# Autodesk Inventor assembly: ASY GBK правая стенка
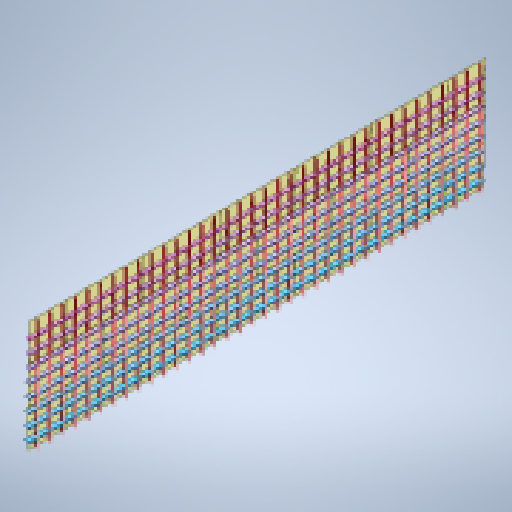
[picture p0: Inventor's stored thumbnail of the model, 512x512]
Saved by Autodesk Inventor 2026.2 (Build 302298000, 298)
## iProperties
Created: 2026-05-20
Part Number: ASY GBK правая стенка
Document SubType Name: Assembly
Designer: admin
Mass: 4.44159e+06 g
Surface Area: 2.86879e+06 cm^2
Volume: 565808 cm^3
Density: 7.85 g/cm^3
Author: admin
## Documents named in this file (6)
- C:\Users\pokla\Documents\Inventor\GBK-Gubkinskiy\ASY GBK правая стенка.iam
- C:\Users\pokla\Documents\Inventor\GBK-Gubkinskiy\ASY GBK 1110 long wall shield 1.iam
- C:\Users\pokla\Documents\Inventor\GBK-Gubkinskiy\ASY GBK 1120 long wall shield 2.iam
- C:\Users\pokla\Documents\Inventor\GBK-Gubkinskiy\ASY GBK 1210 long wall shield 3.iam
- C:\Users\pokla\Documents\Inventor\GBK-Gubkinskiy\ASY GBK 1310 long wall shield 4.iam
- C:\Users\pokla\Documents\Inventor\GBK-Gubkinskiy\ASY GBK 1320 long wall shield 5.iam
## Components (20 placed, 5 different names)
1. ASY GBK 1110 long wall shield 1:1 [sub-assembly] — Flush:1, Mate:1, Mate:2
2. ASY GBK 1120 long wall shield 2:1 [sub-assembly]
3. ASY GBK 1210 long wall shield 3:1 [sub-assembly]
4. ASY GBK 1310 long wall shield 4:1 [sub-assembly]
5. ASY GBK 1320 long wall shield 5:1 [sub-assembly]
6. ASY GBK 1320 long wall shield 5:2 [sub-assembly]
7. ASY GBK 1320 long wall shield 5:3 [sub-assembly]
8. ASY GBK 1320 long wall shield 5:4 [sub-assembly]
9. ASY GBK 1320 long wall shield 5:5 [sub-assembly]
10. ASY GBK 1210 long wall shield 3:2 [sub-assembly]
11. ASY GBK 1210 long wall shield 3:3 [sub-assembly]
12. ASY GBK 1210 long wall shield 3:4 [sub-assembly]
13. ASY GBK 1210 long wall shield 3:5 [sub-assembly]
14. ASY GBK 1210 long wall shield 3:6 [sub-assembly]
15. ASY GBK 1120 long wall shield 2:2 [sub-assembly]
16. ASY GBK 1120 long wall shield 2:3 [sub-assembly]
17. ASY GBK 1120 long wall shield 2:4 [sub-assembly]
18. ASY GBK 1120 long wall shield 2:5 [sub-assembly]
19. ASY GBK 1110 long wall shield 1:2 [sub-assembly]
20. ASY GBK 1310 long wall shield 4:2 [sub-assembly]
## Relationships (22: WeldJoint 19, Mate 2, Flush 1)
- [WeldJoint] (1 mm): ASY GBK 1110 long wall shield 1:1 ↔ ASY GBK 1120 long wall shield 2:1
- [WeldJoint]: ASY GBK 1110 long wall shield 1:1 ↔ ASY GBK 1210 long wall shield 3:1
- [WeldJoint]: ASY GBK 1210 long wall shield 3:1 ↔ ASY GBK 1310 long wall shield 4:1
- [WeldJoint] (1 mm): ASY GBK 1310 long wall shield 4:1 ↔ ASY GBK 1320 long wall shield 5:1
- [WeldJoint] (1 mm): ASY GBK 1320 long wall shield 5:1 ↔ ASY GBK 1320 long wall shield 5:2
- [WeldJoint] (1 mm): ASY GBK 1320 long wall shield 5:2 ↔ ASY GBK 1320 long wall shield 5:3
- [WeldJoint] (1 mm): ASY GBK 1320 long wall shield 5:3 ↔ ASY GBK 1320 long wall shield 5:4
- [WeldJoint] (1 mm): ASY GBK 1320 long wall shield 5:4 ↔ ASY GBK 1320 long wall shield 5:5
- [WeldJoint] (1 mm): ASY GBK 1210 long wall shield 3:1 ↔ ASY GBK 1210 long wall shield 3:2
- [WeldJoint] (1 mm): ASY GBK 1210 long wall shield 3:2 ↔ ASY GBK 1210 long wall shield 3:3
- [WeldJoint] (1 mm): ASY GBK 1210 long wall shield 3:3 ↔ ASY GBK 1210 long wall shield 3:4
- [WeldJoint] (1 mm): ASY GBK 1210 long wall shield 3:4 ↔ ASY GBK 1210 long wall shield 3:5
- [WeldJoint] (1 mm): ASY GBK 1210 long wall shield 3:5 ↔ ASY GBK 1210 long wall shield 3:6
- [WeldJoint] (1 mm): ASY GBK 1120 long wall shield 2:1 ↔ ASY GBK 1120 long wall shield 2:2
- [WeldJoint] (1 mm): ASY GBK 1120 long wall shield 2:2 ↔ ASY GBK 1120 long wall shield 2:3
- [WeldJoint] (1 mm): ASY GBK 1120 long wall shield 2:3 ↔ ASY GBK 1120 long wall shield 2:4
- [WeldJoint] (1 mm): ASY GBK 1120 long wall shield 2:4 ↔ ASY GBK 1120 long wall shield 2:5
- [WeldJoint] (1 mm): ASY GBK 1120 long wall shield 2:5 ↔ ASY GBK 1110 long wall shield 1:2
- [WeldJoint] (1 mm): ASY GBK 1320 long wall shield 5:5 ↔ ASY GBK 1310 long wall shield 4:2
- Flush:1: ASY GBK 1110 long wall shield 1:1
- Mate:1: ASY GBK 1110 long wall shield 1:1
- Mate:2: ASY GBK 1110 long wall shield 1:1
## Named parameters: Зазор_по_горизонту = 1 mm
